# Autodesk Inventor assembly: lamp Assembly
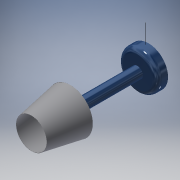
[picture p0: Inventor's stored thumbnail of the model, 180x180]
Saved by Autodesk Inventor 2017 (Build 210142000, 142)
## iProperties
Created: 2017-02-28
Part Number: lamp Assembly
Document SubType Name: Assembly
Designer: Ryan, Jaden, Caleb, Jordan
Engineer: Ryan, Jaden, Caleb, Jordan
Authority: Ryan, Jaden, Caleb, Jordan
Author: Ryan, Jaden, Caleb, Jordan
## Documents named in this file (5)
- C:\Users\rbibb\Desktop\lamp Assembly.iam
- C:\Users\rbibb\AppData\Local\Autodesk\Autodesk Sync\Cloud\rbibby53\S2\Unit 6\Lightbulb-cordair.ipt
- C:\Users\rbibb\Desktop\plug.ipt
- C:\Users\rbibb\Desktop\lam post.ipt
- C:\Users\rbibb\AppData\Local\Autodesk\Autodesk Sync\Cloud\rbibby53\S2\Unit 6\Lamp shade.ipt
## Components (4 placed, 4 different names)
1. Lightbulb-cordair:1 — Mate:1, Cylindrical:1
2. plug:1
3. lam post:1 — Mate:1, Cylindrical:1, Rotational:1
4. Lamp shade:1 — Rotational:1
## Relationships (3: Mate 1, CylindricalJoint 1, RevoluteJoint 1)
- Mate:1: Lightbulb-cordair:1 ↔ lam post:1
- Cylindrical:1: Lightbulb-cordair:1 ↔ lam post:1
- Rotational:1 [RevoluteJoint]: lam post:1 ↔ Lamp shade:1
